# Autodesk Inventor assembly: Endstop Assembly
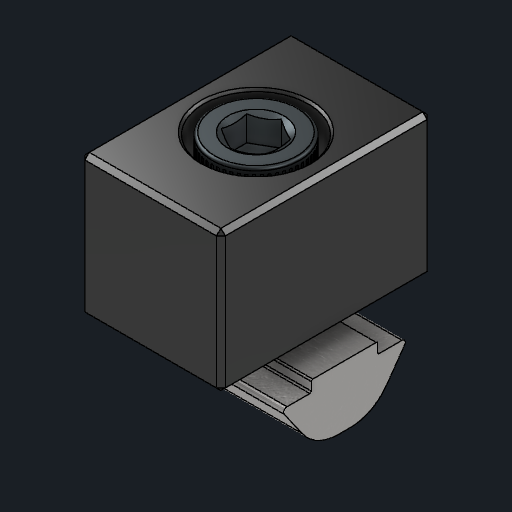
[picture p0: Inventor's stored thumbnail of the model, 512x512]
Saved by Autodesk Inventor 2026.2 (Build 302298000, 298)
## iProperties
Created: 2026-05-18
Part Number: Endstop Assembly
Document SubType Name: Assembly
Designer: JoshuaEah
Author: JoshuaEah
## Documents named in this file (5)
- C:\Users\JoshuaEah\Documents\GitHub\Designed-Trinkets\Modular Pedalboard\Endstop Assembly.iam
- C:\Users\JoshuaEah\Documents\GitHub\Designed-Trinkets\Modular Pedalboard\Fixture Stop.ipt
- C:\Users\JoshuaEah\Documents\GitHub\Designed-Trinkets\Modular Pedalboard\10-32x0.5 SHCS.ipt
- C:\Users\JoshuaEah\Documents\GitHub\Designed-Trinkets\Modular Pedalboard\10-32 T-Nut.ipt
- 10-32 T-Nut.ipt
## Components (3 placed, 3 different names)
1. Fixture Stop:1 — Insert:1
2. 10-32x0.5 SHCS:1 — Insert:1
3. 10-32 T-Nut:1
## Relationships (2: Insert 1, Mate 1)
- Insert:1: Fixture Stop:1 ↔ 10-32x0.5 SHCS:1
- [Mate]: Fixture Stop:1 ↔ 10-32 T-Nut:1
